# Autodesk Inventor assembly: Assembly2
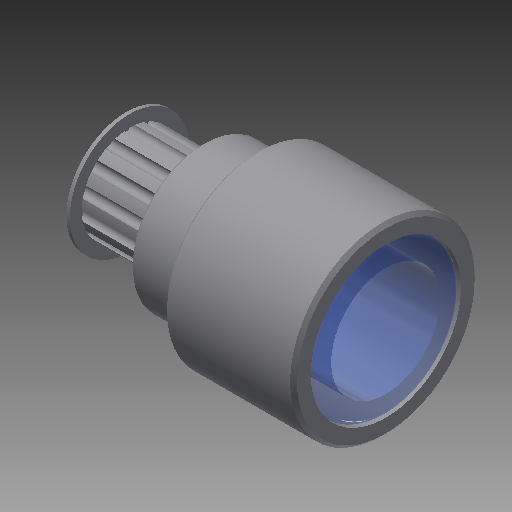
[picture p0: Inventor's stored thumbnail of the model, 512x512]
Saved by Autodesk Inventor 2018.1 (Build 221171000, 171)
## iProperties
Created: 2022-06-29
Part Number: Assembly2
Document SubType Name: Assembly
Designer: Bureau
Author: Bureau
## Documents named in this file (4)
- C:\Users\mouta\GoogleDrive\Manu\USINAGE\MoteurVelo\Arbre secondaire\Assembly2.iam
- C:\Users\mouta\GoogleDrive\Manu\USINAGE\MoteurVelo\Arbre secondaire\roue libre 16 x 22 x 16.ipt
- C:\Users\mouta\GoogleDrive\Manu\USINAGE\MoteurVelo\Arbre secondaire\logement roue libre.ipt
- C:\Users\mouta\GoogleDrive\Manu\USINAGE\MoteurVelo\Arbre secondaire\pignon 15 dents.ipt
## Components (3 placed, 3 different names)
1. roue libre 16 x 22 x 16:1 — Mate:1, Mate:2
2. logement roue libre:1 — Mate:1, Mate:2, Mate:3, Flush:1
3. pignon 15 dents:1 — Mate:3, Flush:1
## Relationships (4: Mate 3, Flush 1)
- Mate:1: roue libre 16 x 22 x 16:1 ↔ logement roue libre:1
- Mate:2: roue libre 16 x 22 x 16:1 ↔ logement roue libre:1
- Mate:3: logement roue libre:1 ↔ pignon 15 dents:1
- Flush:1: logement roue libre:1 ↔ pignon 15 dents:1
